# Autodesk Inventor assembly: V2-Output-Round
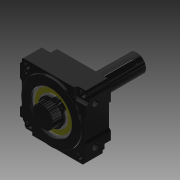
[picture p0: Inventor's stored thumbnail of the model, 180x180]
Saved by Autodesk Inventor 2021 (Build 250183000, 183)
## iProperties
Created: 2018-08-19
Part Number: V2-Output-Round
Document SubType Name: Assembly
Designer: Rafi
Mass: 68.0389 g
Surface Area: 173.636 cm^2
Volume: 32.069 cm^3
Author: Rafi
## Documents named in this file (8)
- E:\Elipse 6814\Elipse Parts Library\Gearboxes\Versaplanetary\V2 Stages\V2 Output Stage\VP V2 Output Stage Round.iam
- E:\Elipse 6814\Elipse Parts Library\Gearboxes\Versaplanetary\V2 Stages\V2 Output Housing.ipt
- E:\Elipse 6814\Elipse Parts Library\Gearboxes\Versaplanetary\V2 Stages\Wave Washer.ipt
- E:\Elipse 6814\Elipse Parts Library\Gearboxes\Versaplanetary\V2 Stages\Retaining Ring.ipt
- E:\Elipse 6814\Elipse Parts Library\Gearboxes\Versaplanetary\Output Shafts\VP 1-2inRound Output.ipt
- E:\Elipse 6814\Elipse Parts Library\Shaft Accessories\Bearings\6902ZZ.ipt
- E:\Elipse 6814\Elipse Parts Library\Shaft Accessories\Bearings.ipt
- E:\Elipse 6814\Elipse Parts Library\Gearboxes\Versaplanetary\V2 Stages\V2 Output Stage.iam
## Components (6 placed, 5 different names)
1. V2 Output Housing:1 — Insert:2, Mate:2, Insert:18
2. 6902ZZ:1 — Insert:2, Insert:23
3. 6902ZZ:2 — Insert:18, Insert:19
4. Wave Washer:1 — Mate:2
5. Retaining Ring:1 — Angle:2, Insert:23
6. VP 1-2inRound Output:1 — Angle:2, Insert:19
## Relationships (6: Insert 4, Mate 1, Angle 1)
- Insert:2: V2 Output Housing:1 ↔ 6902ZZ:1
- Mate:2: V2 Output Housing:1 ↔ Wave Washer:1
- Angle:2 (0 deg): Retaining Ring:1 ↔ VP 1-2inRound Output:1
- Insert:18: V2 Output Housing:1 ↔ 6902ZZ:2
- Insert:19: 6902ZZ:2 ↔ VP 1-2inRound Output:1
- Insert:23 (0.508 mm): 6902ZZ:1 ↔ Retaining Ring:1
